# Autodesk Inventor assembly: modularRICH
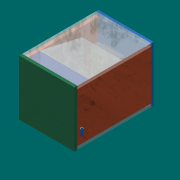
[picture p0: Inventor's stored thumbnail of the model, 180x180]
Saved by Autodesk Inventor 2016 (Build 200138000, 138)
## iProperties
Created: 2015-10-13
Part Number: modularRICH
Document SubType Name: Assembly
Designer: Sawaiz
Author: Sawaiz
## Documents named in this file (9)
- C:\Users\Sawaiz\OneDrive\projects\modularRICH\modularRICH.iam
- C:\Users\Sawaiz\OneDrive\projects\modularRICH\frame\frame.iam
- C:\Users\Sawaiz\OneDrive\projects\modularRICH\aerogelBlock.ipt
- C:\Users\Sawaiz\OneDrive\projects\modularRICH\fresnelLens.ipt
- C:\Users\Sawaiz\OneDrive\projects\modularRICH\mirror\mirrorTopBottom.ipt
- C:\Users\Sawaiz\OneDrive\projects\modularRICH\mirror\mirrorSides.ipt
- C:\Users\Sawaiz\OneDrive\projects\modularRICH\H12700A\H12700A.iam
- C:\Users\Sawaiz\Desktop\91099A167.ipt
- C:\Users\Sawaiz\OneDrive\projects\modularRICH\modularRICH.xlsx
## Components (9 placed, 7 different names)
1. frame:1 [sub-assembly] — Mate:10, Mate:11, Mate:12
2. aerogelBlock:1 — Flush:4, Flush:5, Mate:7, Mate:8, Mate:9, Mate:10, Mate:11, Mate:12
3. fresnelLens:1 — Flush:4, Flush:5, Flush:6, Mate:7
4. mirrorSides:1 — Flush:1, Flush:2, Mate:1, Mate:2, Mate:5, Mate:6, Mate:13
5. mirrorSides:2 — Flush:2, Flush:3, Mate:3, Mate:4, Mate:8
6. mirrorTopBottom:3 — Flush:3, Mate:1, Mate:2, Mate:3, Mate:4, Flush:6
7. mirrorTopBottom:4 — Flush:1, Mate:5, Mate:6, Mate:9
8. H12700A:1 [sub-assembly] — Mate:13
9. 91099A167:1
## Relationships (19: Mate 13, Flush 6)
- Flush:1: mirrorSides:1 ↔ mirrorTopBottom:4
- Flush:2: mirrorSides:1 ↔ mirrorSides:2
- Flush:3: mirrorSides:2 ↔ mirrorTopBottom:3
- Mate:1: mirrorSides:1 ↔ mirrorTopBottom:3
- Mate:2: mirrorSides:1 ↔ mirrorTopBottom:3
- Mate:3: mirrorSides:2 ↔ mirrorTopBottom:3
- Mate:4: mirrorSides:2 ↔ mirrorTopBottom:3
- Mate:5: mirrorSides:1 ↔ mirrorTopBottom:4
- Mate:6: mirrorSides:1 ↔ mirrorTopBottom:4
- Flush:4: aerogelBlock:1 ↔ fresnelLens:1
- Flush:5: aerogelBlock:1 ↔ fresnelLens:1
- Flush:6 (1.624 mm): fresnelLens:1 ↔ mirrorTopBottom:3
- Mate:7: aerogelBlock:1 ↔ fresnelLens:1
- Mate:8: aerogelBlock:1 ↔ mirrorSides:2
- Mate:9: aerogelBlock:1 ↔ mirrorTopBottom:4
- Mate:10: frame:1 ↔ aerogelBlock:1
- Mate:11: frame:1 ↔ aerogelBlock:1
- Mate:12: frame:1 ↔ aerogelBlock:1
- Mate:13: mirrorSides:1 ↔ H12700A:1
## Named parameters: acrylicThickness = 6.35 mm, aerogelThickness = 30 mm, height = 101.6 mm, width = 101.6 mm, depth = 152.4 mm, mirrorAngle = 5 deg, detectorWidth = 52 mm, detectorHeight = 52 mm, mirrorThickness = 3.175 mm, fresnelThickness = 0.1 mm, grooveDensity = 100, focalLength = 76.2 mm, ior = 1.49, centerThickness = 1.524 mm, fresnelAngle = 90 deg, fresnelEffectiveDiameter = 76.2 mm, mirrorSuppourtWidth = 38.1 mm, backGrooveBit = 4.8006 mm, sensorHolderWidth = 88.9 mm, sensorHolderSesnorHeight = 53.975 mm, sensorHolderSensorWidth = 53.975 mm, sensorHolderHeight = 88.9 mm, sensorHolderSensorHeight = 53.975 mm, sensorHolderORingGroove = 3.175 mm, sensorHolderORing = 3.175 mm, sensorHolderFlushORingID = 304.8 mm, sensorHolderFlushORing = 3.175 mm, oRingWidth = 3.175 mm, sensorHolderORingID = 203.2 mm, frontBackORingID = 419.1 mm, topBottomHorizontalMirrorGroove = 12.7 mm, backMirrorGroove = 6.35 mm, mirrorGroove = 19.05 mm, compressionPercent = 40, fresnelChamfer = 6.35 mm, mirrorGrooveFillet = 6.35 mm, mirrorGrooveDrill = 6.35 mm, mirrorGrooveMill = 3.175 mm, fresnelMirrorChamfer = 6.35 mm, detectorOpeningHeight = 76.2 mm, detectorOpeningWidth = 76.2 mm
